# Autodesk Inventor assembly: FullAssembly1
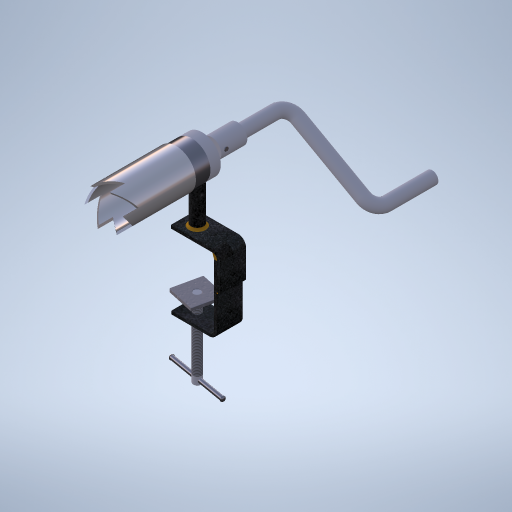
[picture p0: Inventor's stored thumbnail of the model, 512x512]
Saved by Autodesk Inventor 2024.2 (Build 282272000, 272)
## iProperties
Created: 2024-07-01
Part Number: FullAssembly1
Document SubType Name: Assembly
Designer: user
Author: user
## Documents named in this file (9)
- D:\Users\user\Documents\CAD\2024\Maize sheller Version2\FullAssembly1.iam
- D:\Users\user\Documents\CAD\2024\Maize sheller Version2\sleeve.ipt
- D:\Users\user\Documents\CAD\2024\Maize sheller Version2\weldedClampAssembly.iam
- D:\Users\user\Documents\CAD\2024\Maize sheller Version2\shellerAdapter.ipt
- D:\Users\user\Documents\CAD\2024\Maize sheller Version2\FullAssembly1\Design Accelerator\Bearing2.iam
- D:\Users\user\Documents\CAD\2024\Maize sheller Version2\sheller.ipt
- D:\Users\user\Documents\CAD\2024\Maize sheller Version2\handleAdapter.ipt
- D:\Users\user\Documents\CAD\2024\Maize sheller Version2\handle.ipt
- D:\Users\user\Documents\Inventor\Content Center Files\R2024\en-US\BS 1804\BS 1804-2 - 4 x 16.ipt
## Components (8 placed, 8 different names)
1. sleeve:1 — Mate:2, Mate:3, Mate:4, Mate:5, Flush:1, Mate:8
2. weldedClampAssembly:1 [sub-assembly] — Mate:1, Mate:2, Mate:3, Mate:4
3. shellerAdapter:1 — Mate:5, Mate:6, Mate:8, Mate:9, Mate:10, Mate:11, Mate:12, Tangent:1
4. Bearing:1 [sub-assembly] — Mate:6, Mate:7, Rotation:3
5. sheller:1 — Mate:9, Mate:10, Rotation:2
6. handleAdapter:1 — Mate:11, Mate:12, Mate:13, Insert:1, Rotation:1, Rotation:2, Rotation:3, Mate:14
7. handle:1 — Mate:13, Insert:1, Rotation:1
8. BS 1804 : Part 2 4 x 16:1 — Mate:14, Tangent:1
## Relationships (20: Mate 14, RelateRotation 3, Flush 1, Insert 1, Tangent 1)
- Mate:1: weldedClampAssembly:1
- Mate:2: sleeve:1 ↔ weldedClampAssembly:1
- Mate:3 (12.706 mm): sleeve:1 ↔ weldedClampAssembly:1
- Mate:4: sleeve:1 ↔ weldedClampAssembly:1
- Mate:5: sleeve:1 ↔ shellerAdapter:1
- Flush:1 (-2 mm): sleeve:1
- Mate:6: shellerAdapter:1 ↔ Bearing:1
- Mate:7: Bearing:1
- Mate:8: sleeve:1 ↔ shellerAdapter:1
- Mate:9: shellerAdapter:1 ↔ sheller:1
- Mate:10 (-5 mm): shellerAdapter:1 ↔ sheller:1
- Mate:11: shellerAdapter:1 ↔ handleAdapter:1
- Mate:12: shellerAdapter:1 ↔ handleAdapter:1
- Mate:13: handleAdapter:1 ↔ handle:1
- Insert:1: handleAdapter:1 ↔ handle:1
- Rotation:1 [RelateRotation] (1.583 ul): handleAdapter:1 ↔ handle:1
- Rotation:2 [RelateRotation] (2 ul): sheller:1 ↔ handleAdapter:1
- Rotation:3 [RelateRotation] (1.026 ul): Bearing:1 ↔ handleAdapter:1
- Mate:14: handleAdapter:1 ↔ BS 1804 : Part 2 4 x 16:1
- Tangent:1 (-1 mm): shellerAdapter:1 ↔ BS 1804 : Part 2 4 x 16:1
